# Autodesk Inventor assembly: TS_V1_Fallmagazin_Schieber
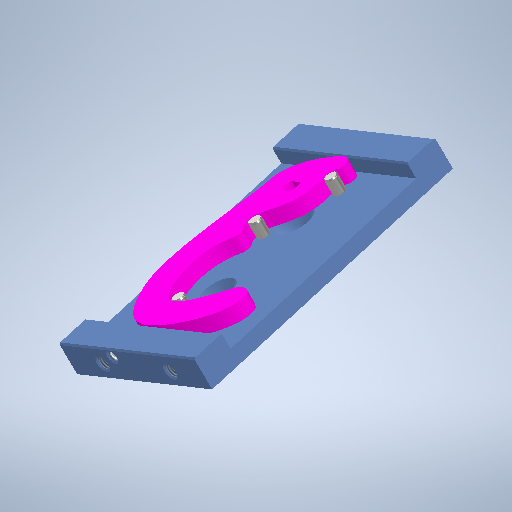
[picture p0: Inventor's stored thumbnail of the model, 512x512]
Saved by Autodesk Inventor 2025.1 (Build 291241000, 241)
## iProperties
Created: 2025-06-11
Part Number: TS_V1_Fallmagazin_Schieber
Document SubType Name: Assembly
Designer: tino
Author: tino
## Documents named in this file (5)
- C:\Users\Erik\Erik\Hochschule\3. Semester\CAD\CAD-Paspa\Useless Box\Eigene Bauteile\Fallmagazin\TS_V1_Fallmagazin_Schieber.iam
- C:\Users\Erik\Erik\Hochschule\3. Semester\CAD\CAD-Paspa\Useless Box\Eigene Bauteile\Fallmagazin\TS_V1_Fallmagazin_Schieber_int.ipt
- C:\Users\Erik\Erik\Hochschule\3. Semester\CAD\CAD-Paspa\Useless Box\_Useless_Box\Finger.ipt
- C:\Users\Erik\Erik\Hochschule\3. Semester\CAD\CAD-Paspa\Useless Box\Kaufteile\WUERTH_federndes_Druckstueck\Wuerth_5099201004_Federndes_Druckstueck,_Kugel,_Edelstahl_LOD_High\Wuerth_5099201004_Federndes_Druckstueck,_Kugel,_.iam
- C:\Users\Erik\Erik\Hochschule\3. Semester\CAD\CAD-Paspa\Useless Box\Standart Bauteile\ISO 2338 - 4 m6 x 8.ipt
## Components (7 placed, 4 different names)
1. TS_V1_Fallmagazin_Schieber_int:1 — Mate:3, Mate:4, Mate:5, Mate:6, Mate:7, Mate:8, Mate:9, Mate:10, Mate:11, Tangent:1, Tangent:2
2. Finger:1 — Mate:3, Tangent:1, Tangent:2, Tangent:3, Tangent:4, Tangent:5, Tangent:6, Tangent:7
3. Wuerth_5099201004_Federndes_Druckstueck,_Kugel,_:1 [sub-assembly] — Mate:5, Tangent:6
4. Wuerth_5099201004_Federndes_Druckstueck,_Kugel,_:2 [sub-assembly] — Mate:4, Tangent:7
5. ISO 2338 4 m6 x 8:1 — Mate:7, Mate:10, Tangent:3
6. ISO 2338 4 m6 x 8:2 — Mate:8, Mate:11, Tangent:4
7. ISO 2338 4 m6 x 8:3 — Mate:6, Mate:9, Tangent:5
## Relationships (16: Mate 9, Tangent 7)
- Mate:3: TS_V1_Fallmagazin_Schieber_int:1 ↔ Finger:1
- Mate:4: TS_V1_Fallmagazin_Schieber_int:1 ↔ Wuerth_5099201004_Federndes_Druckstueck,_Kugel,_:2
- Mate:5: TS_V1_Fallmagazin_Schieber_int:1 ↔ Wuerth_5099201004_Federndes_Druckstueck,_Kugel,_:1
- Mate:6: TS_V1_Fallmagazin_Schieber_int:1 ↔ ISO 2338 4 m6 x 8:3
- Mate:7: TS_V1_Fallmagazin_Schieber_int:1 ↔ ISO 2338 4 m6 x 8:1
- Mate:8: TS_V1_Fallmagazin_Schieber_int:1 ↔ ISO 2338 4 m6 x 8:2
- Mate:9: TS_V1_Fallmagazin_Schieber_int:1 ↔ ISO 2338 4 m6 x 8:3
- Mate:10: TS_V1_Fallmagazin_Schieber_int:1 ↔ ISO 2338 4 m6 x 8:1
- Mate:11: TS_V1_Fallmagazin_Schieber_int:1 ↔ ISO 2338 4 m6 x 8:2
- Tangent:1: TS_V1_Fallmagazin_Schieber_int:1 ↔ Finger:1
- Tangent:2: TS_V1_Fallmagazin_Schieber_int:1 ↔ Finger:1
- Tangent:3: Finger:1 ↔ ISO 2338 4 m6 x 8:1
- Tangent:4: Finger:1 ↔ ISO 2338 4 m6 x 8:2
- Tangent:5: Finger:1 ↔ ISO 2338 4 m6 x 8:3
- Tangent:6: Finger:1 ↔ Wuerth_5099201004_Federndes_Druckstueck,_Kugel,_:1
- Tangent:7: Finger:1 ↔ Wuerth_5099201004_Federndes_Druckstueck,_Kugel,_:2
